# Autodesk Inventor assembly: Module baseplate only
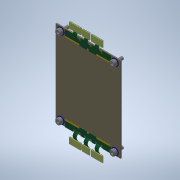
[picture p0: Inventor's stored thumbnail of the model, 180x180]
Saved by Autodesk Inventor 2022 (Build 260153000, 153)
## iProperties
Created: 2021-01-15
Part Number: Module baseplate only
Document SubType Name: Assembly
Designer: caleb
Author: caleb
## Documents named in this file (7)
- C:\Users\Caleb\Desktop\nebraska-silicon-lab\Hardware\ETL\modules\tdr\Module baseplate only.iam
- C:\Users\Caleb\Desktop\nebraska-silicon-lab\Hardware\ETL\modules\tdr\F10109317--_1-MODULE_ CMS2 ETL_ FLEX CIRCUIT.ipt
- C:\Users\Caleb\Desktop\nebraska-silicon-lab\Hardware\ETL\modules\tdr\F10109316--_1-MODULE_ CMS2 ETL_ ALN SUBSTRATE.ipt
- C:\Users\Caleb\Desktop\nebraska-silicon-lab\Hardware\ETL\modules\tdr\F10112323--_1-MODULE_ CMS2 ETL_ FLEX CIRCUIT MOUNTING FILM.ipt
- C:\Users\Caleb\Desktop\nebraska-silicon-lab\Hardware\ETL\modules\tdr\F10110888--_1-MODULE_ CMS2 ETL_ SUBSTRATE MOUNTING THERMAL PAD.ipt
- C:\Users\Caleb\Desktop\nebraska-silicon-lab\Hardware\ETL\modules\tdr\F10109326--_1-WASHER_ BELLEVILLE_ .093IDx.187ODx.01THK_ 17-7 PH STAINLESS STEEL.ipt
- C:\Users\Caleb\Desktop\nebraska-silicon-lab\Hardware\ETL\modules\tdr\FC0041908--_1-SHCS_M2x.4x5LGxFT_SS316L_ROLLED_EP.ipt
## Components (14 placed, 8 different names)
1. F10109317--_1-MODULE_ CMS2 ETL_ FLEX CIRCUIT_1005
2. F10109316--_1-MODULE_ CMS2 ETL_ ALN SUBSTRATE_1006 — Insert:1, Insert:2, Insert:3, Insert:4
3. F10112323--_1-MODULE_ CMS2 ETL_ FLEX CIRCUIT MOUNTING FILM_1011
4. F10110888--_1-MODULE_ CMS2 ETL_ SUBSTRATE MOUNTING THERMAL PAD_1012
5. F10109317--_1-MODULE_ CMS2 ETL_ FLEX CIRCUIT_1013
6. F10112323--_1-MODULE_ CMS2 ETL_ FLEX CIRCUIT MOUNTING FILM_1014
7. F10109326--_1-WASHER_ BELLEVILLE_ .093IDx.187ODx.01THK_ 17-7 PH STAINLESS STEEL:1 — Insert:2, Insert:7
8. F10109326--_1-WASHER_ BELLEVILLE_ .093IDx.187ODx.01THK_ 17-7 PH STAINLESS STEEL:2 — Insert:4, Insert:5
9. F10109326--_1-WASHER_ BELLEVILLE_ .093IDx.187ODx.01THK_ 17-7 PH STAINLESS STEEL:3 — Insert:3, Insert:8
10. F10109326--_1-WASHER_ BELLEVILLE_ .093IDx.187ODx.01THK_ 17-7 PH STAINLESS STEEL:4 — Insert:1, Insert:6
11. FC0041908--_1-SHCS_M2x.4x5LGxFT_SS316L_ROLLED_EP:1 — Insert:5
12. FC0041908--_1-SHCS_M2x.4x5LGxFT_SS316L_ROLLED_EP:2 — Insert:6
13. FC0041908--_1-SHCS_M2x.4x5LGxFT_SS316L_ROLLED_EP:3 — Insert:7
14. FC0041908--_1-SHCS_M2x.4x5LGxFT_SS316L_ROLLED_EP:4 — Insert:8
## Relationships (8: Insert 8)
- Insert:1: F10109316--_1-MODULE_ CMS2 ETL_ ALN SUBSTRATE_1006 ↔ F10109326--_1-WASHER_ BELLEVILLE_ .093IDx.187ODx.01THK_ 17-7 PH STAINLESS STEEL:4
- Insert:2: F10109316--_1-MODULE_ CMS2 ETL_ ALN SUBSTRATE_1006 ↔ F10109326--_1-WASHER_ BELLEVILLE_ .093IDx.187ODx.01THK_ 17-7 PH STAINLESS STEEL:1
- Insert:3: F10109316--_1-MODULE_ CMS2 ETL_ ALN SUBSTRATE_1006 ↔ F10109326--_1-WASHER_ BELLEVILLE_ .093IDx.187ODx.01THK_ 17-7 PH STAINLESS STEEL:3
- Insert:4: F10109316--_1-MODULE_ CMS2 ETL_ ALN SUBSTRATE_1006 ↔ F10109326--_1-WASHER_ BELLEVILLE_ .093IDx.187ODx.01THK_ 17-7 PH STAINLESS STEEL:2
- Insert:5: F10109326--_1-WASHER_ BELLEVILLE_ .093IDx.187ODx.01THK_ 17-7 PH STAINLESS STEEL:2 ↔ FC0041908--_1-SHCS_M2x.4x5LGxFT_SS316L_ROLLED_EP:1
- Insert:6: F10109326--_1-WASHER_ BELLEVILLE_ .093IDx.187ODx.01THK_ 17-7 PH STAINLESS STEEL:4 ↔ FC0041908--_1-SHCS_M2x.4x5LGxFT_SS316L_ROLLED_EP:2
- Insert:7: F10109326--_1-WASHER_ BELLEVILLE_ .093IDx.187ODx.01THK_ 17-7 PH STAINLESS STEEL:1 ↔ FC0041908--_1-SHCS_M2x.4x5LGxFT_SS316L_ROLLED_EP:3
- Insert:8: F10109326--_1-WASHER_ BELLEVILLE_ .093IDx.187ODx.01THK_ 17-7 PH STAINLESS STEEL:3 ↔ FC0041908--_1-SHCS_M2x.4x5LGxFT_SS316L_ROLLED_EP:4
